# Autodesk Inventor assembly: Assembly-Whole
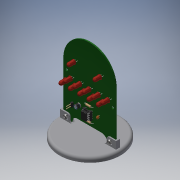
[picture p0: Inventor's stored thumbnail of the model, 180x180]
Saved by Autodesk Inventor 2018 (Build 220112000, 112)
## iProperties
Created: 2019-08-28
Part Number: Assembly-Whole
Document SubType Name: Assembly
Designer: Electro707
Author: Electro707
## Documents named in this file (5)
- F:\Projects\UNH MakerSpace Kits\2019 - Halloween Event\Ghost\GitHub Folder\CAD-Inventor\Assembly-Whole.iam
- F:\Projects\UNH MakerSpace Kits\2019 - Halloween Event\Ghost\GitHub Folder\CAD-Inventor\Assembly-PCB Alone.iam
- F:\Projects\UNH MakerSpace Kits\2019 - Halloween Event\Ghost\GitHub Folder\CAD-Inventor\Base.ipt
- F:\Projects\UNH MakerSpace Kits\2019 - Halloween Event\Ghost\GitHub Folder\CAD-Inventor\ANSI B18.6.7M - M3x0.5 x 8(4).ipt
- F:\Projects\UNH MakerSpace Kits\2019 - Halloween Event\Ghost\GitHub Folder\CAD-Inventor\ANSI B 18.2.4.1 M - M3 x 0.5Style 1.ipt
## Components (6 placed, 4 different names)
1. Assembly-PCB Alone:1 [sub-assembly] — Mate:1, Mate:2, Mate:11, Mate:12
2. Base:1 — Mate:1, Mate:2, Mate:3, Mate:4, Mate:5, Mate:6, Mate:7, Mate:8, Mate:9, Mate:10, Mate:13, Mate:14
3. ANSI B18.6.7M - M3x0.5 x 8(4):1 — Mate:3, Mate:6
4. ANSI B18.6.7M - M3x0.5 x 8(4):2 — Mate:4, Mate:5
5. ANSI B 18.2.4.1 M - M3 x 0.5Style 1:1 — Mate:8, Mate:9, Mate:18, Mate:19
6. ANSI B 18.2.4.1 M - M3 x 0.5Style 1:2 — Mate:7, Mate:10, Mate:16, Mate:17
## Relationships (20: Mate 20)
- Mate:1: Assembly-PCB Alone:1 ↔ Base:1
- Mate:2: Assembly-PCB Alone:1 ↔ Base:1
- Mate:3: Base:1 ↔ ANSI B18.6.7M - M3x0.5 x 8(4):1
- Mate:4: Base:1 ↔ ANSI B18.6.7M - M3x0.5 x 8(4):2
- Mate:5: Base:1 ↔ ANSI B18.6.7M - M3x0.5 x 8(4):2
- Mate:6: Base:1 ↔ ANSI B18.6.7M - M3x0.5 x 8(4):1
- Mate:7: Base:1 ↔ ANSI B 18.2.4.1 M - M3 x 0.5Style 1:2
- Mate:8: Base:1 ↔ ANSI B 18.2.4.1 M - M3 x 0.5Style 1:1
- Mate:9: Base:1 ↔ ANSI B 18.2.4.1 M - M3 x 0.5Style 1:1
- Mate:10: Base:1 ↔ ANSI B 18.2.4.1 M - M3 x 0.5Style 1:2
- Mate:11: Assembly-PCB Alone:1
- Mate:12: Assembly-PCB Alone:1
- Mate:13: Base:1
- Mate:14: Base:1
- Mate:15
- Mate:16: ANSI B 18.2.4.1 M - M3 x 0.5Style 1:2
- Mate:17: ANSI B 18.2.4.1 M - M3 x 0.5Style 1:2
- Mate:18: ANSI B 18.2.4.1 M - M3 x 0.5Style 1:1
- Mate:19: ANSI B 18.2.4.1 M - M3 x 0.5Style 1:1
- Mate:20
